# Autodesk Inventor assembly: Motor Assembly
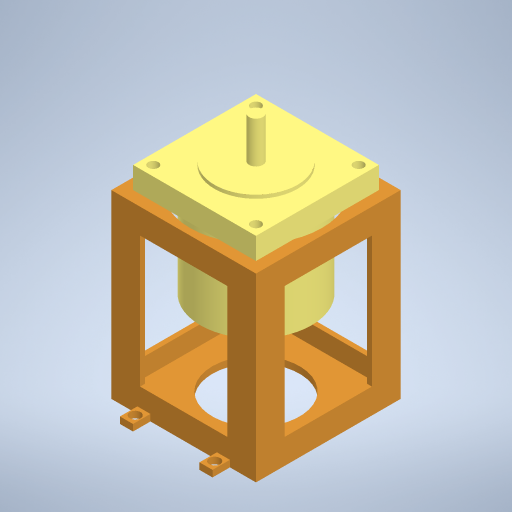
[picture p0: Inventor's stored thumbnail of the model, 512x512]
Saved by Autodesk Inventor 2023 (Build 270158000, 158)
## iProperties
Created: 2023-02-22
Part Number: Motor Assembly
Document SubType Name: Assembly
Designer: cheng
Author: cheng
## Documents named in this file (3)
- C:\Users\mihal\Desktop\4th Year Project\Final Assembly\Motor Casing\Motor Assembly.iam
- C:\Users\mihal\Desktop\4th Year Project\Final Assembly\Motor Casing\Motor case.ipt
- C:\Users\mihal\Desktop\4th Year Project\Final Assembly\Motor Casing\Motor model.ipt
## Components (2 placed, 2 different names)
1. Motor case:1 — Mate:1, Mate:2, Mate:4
2. Motor model:1 — Mate:1, Mate:2, Mate:4
## Relationships (3: Mate 3)
- Mate:1: Motor case:1 ↔ Motor model:1
- Mate:2: Motor case:1 ↔ Motor model:1
- Mate:4: Motor case:1 ↔ Motor model:1
